# Autodesk Inventor assembly: ABD_Version_0.1_leftleg
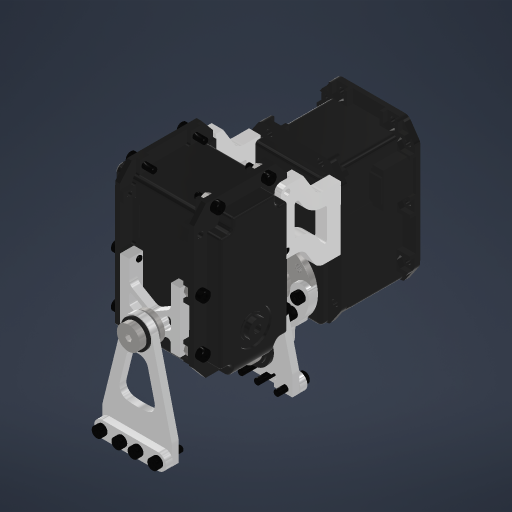
[picture p0: Inventor's stored thumbnail of the model, 512x512]
Saved by Autodesk Inventor 2024.3 (Build 283343000, 343)
## iProperties
Created: 2024-01-23
Part Number: ABD_Version_0.1_leftleg
Document SubType Name: Assembly
Designer: ASUS
Mass: 357.136 g
Surface Area: 604.848 cm^2
Volume: 181.423 cm^3
Density: 1.96853 g/cm^3
Author: ASUS
## Documents named in this file (17)
- C:\Users\ASUS\Desktop\Anti_Backlash_Structure_OP\v4_Frame\ABD_V4_Left_OP.iam
- C:\Users\ASUS\Desktop\Anti_Backlash_Structure_OP\v4_Frame\ABD_MX_64_Roll_Fixation_Set.iam
- C:\Users\ASUS\Desktop\Anti_Backlash_Structure_OP\v4_Frame\ABD_Slider_Set_v4.iam
- C:\Users\ASUS\Desktop\Anti_Backlash_Structure_OP\MISUMI\C-WSSA12-4-2.ipt
- C:\Users\ASUS\Desktop\Anti_Backlash_Structure_OP\MISUMI\NBW-0612-10.ipt
- C:\Users\ASUS\Desktop\Anti_Backlash_Structure_OP\MISUMI\LED-0606.ipt
- C:\Users\ASUS\Desktop\Anti_Backlash_Structure_OP\v4_Frame\Ubber_Washer_1.5mm.ipt
- C:\Users\ASUS\Desktop\Anti_Backlash_Structure_OP\MISUMI\DBB4-8-5.ipt
- C:\Users\ASUS\Desktop\Anti_Backlash_Structure_OP\v4_Frame\Roll_Fixation_Frame.ipt
- C:\Users\ASUS\Desktop\Anti_Backlash_Structure_OP\v4_Frame\Roll_Fixation_Frame_Back.ipt
- C:\Users\ASUS\Desktop\Anti_Backlash_Structure_OP\v4_Frame\hip joint fix washer.ipt
- C:\Users\ASUS\Desktop\Anti_Backlash_Structure_OP\MISUMI\hip_joint_fix_washer_10mm_Set.iam
- C:\Users\ASUS\Desktop\Anti_Backlash_Structure_OP\v4_Frame\Front_Frame_Fixer_v2.iam
- C:\Users\ASUS\Desktop\Anti_Backlash_Structure_OP\ROBOTIS(Inventor 2024 ver.)\DXL\MX-64T.ipt
- C:\Users\ASUS\Desktop\Anti_Backlash_Structure_OP\MISUMI\DBSY4-5-8.ipt
- C:\Users\ASUS\Desktop\Anti_Backlash_Structure_OP\v4_Frame\Dynamixel Vertical fixation.ipt
- C:\Users\ASUS\Desktop\Anti_Backlash_Structure_OP\v4_Frame\Dynamixel Vertical fixation_MIR.ipt
## Components (21 placed, 16 different names)
1. Roll_Fixation_Frame:1
2. hip joint fix washer:1
3. hip joint fix washer:2 — 삽입:47, 메이트:29
4. hip_joint_fix_washer_10mm_Set:1 [sub-assembly]
5. hip_joint_fix_washer_10mm_Set:2 [sub-assembly] — 메이트:29
6. Front_Frame_Fixer_v2:1 [sub-assembly] — 삽입:46
7. DBSY4-5-8:1
8. ABD_MX_64_Roll_Fixation_Set:2 [sub-assembly] — 각도:3, 플러쉬:1, 삽입:46, 삽입:49, 삽입:52
9. MX-64T:1 — 삽입:43, 각도:3, 플러쉬:1, 메이트:30, 메이트:31, 메이트:32, 삽입:48, 메이트:33, 각도:4
10. LED-0606:2 — 메이트:34
11. Ubber_Washer_1.5mm:2 — 메이트:28
12. DBB4-8-5:2
13. NBW-0612-10:3
14. C-WSSA12-4-2:2
15. NBW-0612-10:4
16. ABD_Slider_Set_v4:2 [sub-assembly] — 삽입:43
17. Roll_Fixation_Frame_Back:3 — 메이트:28, 삽입:47, 메이트:34, 삽입:51, 각도:4
18. Dynamixel Vertical fixation:1 — 메이트:30, 메이트:31, 메이트:32
19. Dynamixel Vertical fixation_MIR:1 — 삽입:48, 메이트:33, 삽입:49
20. Front_Frame_Fixer_v2:2 [sub-assembly] — 삽입:51, 삽입:52
21. DBSY4-5-8:2
## Relationships (36: Insert 20, Mate 13, Angle 2, Flush 1)
- [Insert]: Roll_Fixation_Frame:1 ↔ hip joint fix washer:1
- [Insert]: Roll_Fixation_Frame:1 ↔ hip joint fix washer:1
- [Mate]: Roll_Fixation_Frame:1 ↔ hip joint fix washer:1
- [Insert]: hip joint fix washer:1 ↔ hip_joint_fix_washer_10mm_Set:1
- [Mate]: hip joint fix washer:1 ↔ hip_joint_fix_washer_10mm_Set:1
- [Insert]: hip joint fix washer:2 ↔ hip_joint_fix_washer_10mm_Set:2
- [Mate]: hip joint fix washer:2 ↔ hip_joint_fix_washer_10mm_Set:2
- [Mate]: hip_joint_fix_washer_10mm_Set:1 ↔ hip_joint_fix_washer_10mm_Set:2
- [Mate]: hip_joint_fix_washer_10mm_Set:1 ↔ hip_joint_fix_washer_10mm_Set:2
- [Insert]: Front_Frame_Fixer_v2:1 ↔ DBSY4-5-8:1
- [Insert]: Roll_Fixation_Frame:1 ↔ Front_Frame_Fixer_v2:1
- [Insert]: LED-0606:2 ↔ Ubber_Washer_1.5mm:2
- [Insert]: Ubber_Washer_1.5mm:2 ↔ NBW-0612-10:4
- [Insert]: DBB4-8-5:2 ↔ NBW-0612-10:4
- [Insert]: NBW-0612-10:3 ↔ C-WSSA12-4-2:2
- [Mate]: DBB4-8-5:2 ↔ ABD_Slider_Set_v4:2
- [Insert]: LED-0606:2 ↔ NBW-0612-10:3
- [Insert]: C-WSSA12-4-2:2 ↔ ABD_Slider_Set_v4:2
- 삽입:43 [Insert] (0.5 mm): MX-64T:1 ↔ ABD_Slider_Set_v4:2
- 각도:3 [Angle] (0 deg): ABD_MX_64_Roll_Fixation_Set:2 ↔ MX-64T:1
- 플러쉬:1 [Flush] (-3.1 mm): ABD_MX_64_Roll_Fixation_Set:2 ↔ MX-64T:1
- 메이트:28 [Mate]: Ubber_Washer_1.5mm:2 ↔ Roll_Fixation_Frame_Back:3
- 삽입:46 [Insert]: Front_Frame_Fixer_v2:1 ↔ ABD_MX_64_Roll_Fixation_Set:2
- 삽입:47 [Insert]: hip joint fix washer:2 ↔ Roll_Fixation_Frame_Back:3
- 메이트:29 [Mate]: hip joint fix washer:2 ↔ hip_joint_fix_washer_10mm_Set:2
- 메이트:30 [Mate]: MX-64T:1 ↔ Dynamixel Vertical fixation:1
- 메이트:31 [Mate]: MX-64T:1 ↔ Dynamixel Vertical fixation:1
- 메이트:32 [Mate]: MX-64T:1 ↔ Dynamixel Vertical fixation:1
- 삽입:48 [Insert]: MX-64T:1 ↔ Dynamixel Vertical fixation_MIR:1
- 메이트:33 [Mate]: MX-64T:1 ↔ Dynamixel Vertical fixation_MIR:1
- 삽입:49 [Insert] (0.05 mm): ABD_MX_64_Roll_Fixation_Set:2 ↔ Dynamixel Vertical fixation_MIR:1
- 메이트:34 [Mate] (0.5 mm): LED-0606:2 ↔ Roll_Fixation_Frame_Back:3
- [Insert]: Front_Frame_Fixer_v2:2 ↔ DBSY4-5-8:2
- 삽입:51 [Insert]: Roll_Fixation_Frame_Back:3 ↔ Front_Frame_Fixer_v2:2
- 삽입:52 [Insert]: ABD_MX_64_Roll_Fixation_Set:2 ↔ Front_Frame_Fixer_v2:2
- 각도:4 [Angle] (0 deg): MX-64T:1 ↔ Roll_Fixation_Frame_Back:3
## Named parameters: d1010_d968 = 0 mm, d1011_d969 = 0 mm, d1012_d971 = 0 mm, d1013_d941 = 0 mm, d1014_d956 = 0 mm, d1015_d957 = 0 mm, d1016_d960 = 0 mm, d1047_d49 = 0 mm
